# Autodesk Inventor assembly: wheel
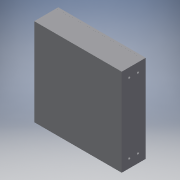
[picture p0: Inventor's stored thumbnail of the model, 180x180]
Saved by Autodesk Inventor 2018 (Build 220112000, 112)
## iProperties
Created: 2018-08-07
Part Number: wheel
Document SubType Name: Assembly
Designer: Cole Tucker
Author: Cole Tucker
## Documents named in this file (3)
- C:\Users\Cole Tucker\OneDrive\FRC-mxpProject\Cad\steering\wheel.iam
- C:\Users\Cole Tucker\OneDrive\FRC-mxpProject\Cad\steering\wheel core.ipt
- C:\Users\Cole Tucker\OneDrive\FRC-mxpProject\Cad\steering\wheel coreBack.ipt
## Components (2 placed, 2 different names)
1. wheel core:1 — Mate:1, Flush:1, Flush:2
2. wheel coreBack:1 — Mate:1, Flush:1, Flush:2
## Relationships (3: Flush 2, Mate 1)
- Mate:1: wheel core:1 ↔ wheel coreBack:1
- Flush:1: wheel core:1 ↔ wheel coreBack:1
- Flush:2: wheel core:1 ↔ wheel coreBack:1
